# Autodesk Inventor assembly: Julie
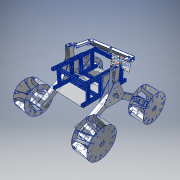
[picture p0: Inventor's stored thumbnail of the model, 180x180]
Saved by Autodesk Inventor 2019 (Build 230136000, 136)
## iProperties
Created: 2018-09-27
Part Number: Julie
Document SubType Name: Assembly
Designer: Adhik
Mass: 21285.8 g
Surface Area: 63277.1 cm^2
Volume: 8790.97 cm^3
Density: 2.42133 g/cm^3
Author: Adhik
## Documents named in this file (19)
- C:\Users\Adhik\Documents\CAD\Julie\Julie.iam
- C:\Users\Adhik\Documents\CAD\Julie\Baseplate.ipt
- C:\Users\Adhik\Documents\CAD\Julie\Lateral Plate.ipt
- C:\Users\Adhik\Documents\CAD\Julie\Right Drive Assembly.iam
- C:\Users\Adhik\Documents\CAD\Julie\Main Joint.ipt
- C:\Users\Adhik\Documents\CAD\Julie\8020 20 inch lower.ipt
- C:\Users\Adhik\Documents\CAD\Julie\8020 6 inch.ipt
- C:\Users\Adhik\Documents\CAD\Julie\Main Axle.ipt
- C:\Users\Adhik\Documents\CAD\Julie\8020 12 inch.ipt
- C:\Users\Adhik\Documents\CAD\Julie\Clamp Collar.ipt
- C:\Users\Adhik\Documents\CAD\Julie\Coupler.ipt
- C:\Users\Adhik\Documents\CAD\Julie\Crossbeam Bearing Mount.ipt
- C:\Users\Adhik\Documents\CAD\Julie\Joint Mount.ipt
- C:\Users\Adhik\Documents\CAD\Julie\Ball Joint.ipt
- C:\Users\Adhik\Documents\CAD\Julie\Crossbeam.ipt
- C:\Users\Adhik\Documents\CAD\Julie\Crossbeam Post.ipt
- C:\Users\Adhik\Documents\CAD\Julie\Front Cover.ipt
- C:\Users\Adhik\Documents\CAD\Julie\Rear Cover.ipt
- C:\Users\Adhik\Documents\CAD\Julie\8020 20 inch upper.ipt
## Components (40 placed, 18 different names)
1. Baseplate:1 — Flush:5, Flush:6, Mate:13, Mate:14, Mate:15, Mate:16, Mate:35, Mate:36, Flush:34, Flush:35
2. Lateral Plate:1 — Flush:5, Mate:5, Mate:7, Mate:8, Mate:14, Mate:18, Mate:23, Mate:24, Mate:86, Mate:87, Mate:88, Mate:89, Flush:28, Flush:30, Flush:31
3. Lateral Plate:2 — Flush:6, Mate:6, Mate:9, Mate:10, Mate:13, Mate:17, Mate:21, Mate:22, Flush:27, Flush:32, Flush:33
4. Right Drive Assembly:2 [sub-assembly] — Mate:11, Mate:34, Mate:50, Mate:58, Mate:60, Mate:61
5. Main Joint:1 — Mate:5, Mate:7, Mate:8, Mate:56
6. Main Joint:2 — Mate:6, Mate:9, Mate:10, Mate:11, Mate:32, Mate:34
7. 8020 20 inch lower:1 — Mate:15, Mate:17, Mate:25, Mate:26, Mate:37, Mate:39, Mate:90, Flush:23, Mate:91, Flush:24, Flush:35, Flush:36
8. 8020 20 inch lower:2 — Mate:16, Mate:18, Mate:27, Mate:28, Mate:92, Mate:93, Flush:25, Flush:26, Flush:34, Flush:39
9. 8020 6 inch:1 — Mate:21, Mate:25, Mate:46, Mate:98, Flush:37
10. 8020 6 inch:2 — Mate:22, Mate:26, Mate:44
11. 8020 6 inch:3 — Mate:24, Mate:27
12. 8020 6 inch:4 — Mate:23, Mate:28, Flush:38, Mate:99
13. Main Axle:1 — Mate:31, Mate:32, Mate:48, Mate:49, Mate:55
14. 8020 12 inch:1 — Mate:35, Mate:37
15. 8020 12 inch:2 — Mate:36, Mate:39, Mate:97
16. 8020 12 inch:3 — Mate:44, Mate:53, Mate:54, Flush:21, Flush:22, Mate:101
17. 8020 12 inch:4 — Mate:46, Flush:40, Mate:100
18. Clamp Collar:1 — Mate:48, Mate:50
19. Clamp Collar:2 — Mate:49, Mate:57
20. Coupler:1 — Mate:72, Mate:79
21. Coupler:2 — Mate:71, Mate:78
22. Crossbeam Bearing Mount:1 — Mate:53, Flush:19, Flush:21, Mate:95, Mate:96
23. Crossbeam Bearing Mount:2 — Mate:54, Flush:20, Flush:22
24. Right Drive Assembly:3 [sub-assembly] — Mate:55, Mate:56, Mate:57, Mate:59, Mate:62, Mate:63
25. Joint Mount:1 — Mate:59, Mate:62, Mate:63, Mate:64, Mate:68, Mate:69
26. Joint Mount:2 — Mate:58, Mate:60, Mate:61, Mate:65, Mate:67, Mate:70
27. Ball Joint:1 — Mate:64, Mate:68, Mate:69, Mate:71
28. Ball Joint:2 — Mate:65, Mate:67, Mate:70, Mate:72
29. Crossbeam:1 — Mate:74, Mate:75, Mate:76, Mate:77, Mate:80, Mate:81, Mate:94, Mate:96
30. Ball Joint:3 — Mate:75, Mate:76, Mate:79, Mate:80
31. Ball Joint:4 — Mate:74, Mate:77, Mate:78, Mate:81
32. Crossbeam Post:1 — Mate:94, Mate:95
33. Front Cover:1 — Mate:86, Mate:87
34. Rear Cover:1 — Mate:88, Mate:89
35. 8020 6 inch:5 — Mate:90, Flush:23, Flush:32
36. 8020 6 inch:6 — Mate:92, Flush:26, Mate:97, Flush:30
37. 8020 6 inch:8 — Mate:93, Flush:25, Flush:31
38. 8020 6 inch:9 — Mate:91, Flush:24, Flush:33
39. 8020 20 inch upper:1 — Flush:36, Mate:98, Flush:37, Flush:40, Mate:100
40. 8020 20 inch upper:2 — Flush:38, Mate:99, Flush:39, Mate:101
## Relationships (99: Mate 76, Flush 23)
- Flush:5: Baseplate:1 ↔ Lateral Plate:1
- Flush:6: Baseplate:1 ↔ Lateral Plate:2
- Mate:5: Lateral Plate:1 ↔ Main Joint:1
- Mate:6: Lateral Plate:2 ↔ Main Joint:2
- Mate:7: Lateral Plate:1 ↔ Main Joint:1
- Mate:8: Lateral Plate:1 ↔ Main Joint:1
- Mate:9: Lateral Plate:2 ↔ Main Joint:2
- Mate:10: Lateral Plate:2 ↔ Main Joint:2
- Mate:11: Right Drive Assembly:2 ↔ Main Joint:2
- Mate:13: Baseplate:1 ↔ Lateral Plate:2
- Mate:14: Baseplate:1 ↔ Lateral Plate:1
- Mate:15: Baseplate:1 ↔ 8020 20 inch lower:1
- Mate:16: Baseplate:1 ↔ 8020 20 inch lower:2
- Mate:17: Lateral Plate:2 ↔ 8020 20 inch lower:1
- Mate:18: Lateral Plate:1 ↔ 8020 20 inch lower:2
- Mate:21: Lateral Plate:2 ↔ 8020 6 inch:1
- Mate:22: Lateral Plate:2 ↔ 8020 6 inch:2
- Mate:23: Lateral Plate:1 ↔ 8020 6 inch:4
- Mate:24: Lateral Plate:1 ↔ 8020 6 inch:3
- Mate:25: 8020 20 inch lower:1 ↔ 8020 6 inch:1
- Mate:26: 8020 20 inch lower:1 ↔ 8020 6 inch:2
- Mate:27: 8020 20 inch lower:2 ↔ 8020 6 inch:3
- Mate:28: 8020 20 inch lower:2 ↔ 8020 6 inch:4
- Mate:31: Main Axle:1
- Mate:32: Main Joint:2 ↔ Main Axle:1
- Mate:34: Right Drive Assembly:2 ↔ Main Joint:2
- Mate:35: Baseplate:1 ↔ 8020 12 inch:1
- Mate:36: Baseplate:1 ↔ 8020 12 inch:2
- Mate:37: 8020 20 inch lower:1 ↔ 8020 12 inch:1
- Mate:39: 8020 20 inch lower:1 ↔ 8020 12 inch:2
- Mate:44: 8020 6 inch:2 ↔ 8020 12 inch:3
- Mate:46: 8020 6 inch:1 ↔ 8020 12 inch:4
- Mate:48: Main Axle:1 ↔ Clamp Collar:1
- Mate:49: Main Axle:1 ↔ Clamp Collar:2
- Mate:50: Right Drive Assembly:2 ↔ Clamp Collar:1
- Mate:53: 8020 12 inch:3 ↔ Crossbeam Bearing Mount:1
- Mate:54: 8020 12 inch:3 ↔ Crossbeam Bearing Mount:2
- Flush:19: Crossbeam Bearing Mount:1
- Flush:20: Crossbeam Bearing Mount:2
- Flush:21: 8020 12 inch:3 ↔ Crossbeam Bearing Mount:1
- Flush:22: 8020 12 inch:3 ↔ Crossbeam Bearing Mount:2
- Mate:55: Main Axle:1 ↔ Right Drive Assembly:3
- Mate:56: Main Joint:1 ↔ Right Drive Assembly:3
- Mate:57: Clamp Collar:2 ↔ Right Drive Assembly:3
- Mate:58: Right Drive Assembly:2 ↔ Joint Mount:2
- Mate:59: Right Drive Assembly:3 ↔ Joint Mount:1
- Mate:60: Right Drive Assembly:2 ↔ Joint Mount:2
- Mate:61: Right Drive Assembly:2 ↔ Joint Mount:2
- Mate:62: Right Drive Assembly:3 ↔ Joint Mount:1
- Mate:63: Right Drive Assembly:3 ↔ Joint Mount:1
- Mate:64: Joint Mount:1 ↔ Ball Joint:1
- Mate:65: Joint Mount:2 ↔ Ball Joint:2
- Mate:67: Joint Mount:2 ↔ Ball Joint:2
- Mate:68: Joint Mount:1 ↔ Ball Joint:1
- Mate:69: Joint Mount:1 ↔ Ball Joint:1
- Mate:70: Joint Mount:2 ↔ Ball Joint:2
- Mate:71: Coupler:2 ↔ Ball Joint:1
- Mate:72: Coupler:1 ↔ Ball Joint:2
- Mate:74: Crossbeam:1 ↔ Ball Joint:4
- Mate:75: Crossbeam:1 ↔ Ball Joint:3
- Mate:76: Crossbeam:1 ↔ Ball Joint:3
- Mate:77: Crossbeam:1 ↔ Ball Joint:4
- Mate:78: Coupler:2 ↔ Ball Joint:4
- Mate:79: Coupler:1 ↔ Ball Joint:3
- Mate:80: Crossbeam:1 ↔ Ball Joint:3
- Mate:81: Crossbeam:1 ↔ Ball Joint:4
- Mate:86: Lateral Plate:1 ↔ Front Cover:1
- Mate:87: Lateral Plate:1 ↔ Front Cover:1
- Mate:88: Lateral Plate:1 ↔ Rear Cover:1
- Mate:89: Lateral Plate:1 ↔ Rear Cover:1
- Mate:90: 8020 20 inch lower:1 ↔ 8020 6 inch:5
- Flush:23: 8020 20 inch lower:1 ↔ 8020 6 inch:5
- Mate:91: 8020 20 inch lower:1 ↔ 8020 6 inch:9
- Flush:24: 8020 20 inch lower:1 ↔ 8020 6 inch:9
- Mate:92: 8020 20 inch lower:2 ↔ 8020 6 inch:6
- Mate:93: 8020 20 inch lower:2 ↔ 8020 6 inch:8
- Flush:25: 8020 20 inch lower:2 ↔ 8020 6 inch:8
- Flush:26: 8020 20 inch lower:2 ↔ 8020 6 inch:6
- Mate:94: Crossbeam:1 ↔ Crossbeam Post:1
- Mate:95: Crossbeam Bearing Mount:1 ↔ Crossbeam Post:1
- Flush:27: Lateral Plate:2
- Flush:28: Lateral Plate:1
- Mate:96 (12.7 mm): Crossbeam Bearing Mount:1 ↔ Crossbeam:1
- Mate:97: 8020 12 inch:2 ↔ 8020 6 inch:6
- Flush:30: Lateral Plate:1 ↔ 8020 6 inch:6
- Flush:31: Lateral Plate:1 ↔ 8020 6 inch:8
- Flush:32: Lateral Plate:2 ↔ 8020 6 inch:5
- Flush:33: Lateral Plate:2 ↔ 8020 6 inch:9
- Flush:34: Baseplate:1 ↔ 8020 20 inch lower:2
- Flush:35: Baseplate:1 ↔ 8020 20 inch lower:1
- Flush:36: 8020 20 inch lower:1 ↔ 8020 20 inch upper:1
- Mate:98: 8020 6 inch:1 ↔ 8020 20 inch upper:1
- Flush:37: 8020 6 inch:1 ↔ 8020 20 inch upper:1
- Flush:38: 8020 6 inch:4 ↔ 8020 20 inch upper:2
- Mate:99: 8020 6 inch:4 ↔ 8020 20 inch upper:2
- Flush:39: 8020 20 inch lower:2 ↔ 8020 20 inch upper:2
- Flush:40: 8020 12 inch:4 ↔ 8020 20 inch upper:1
- Mate:100: 8020 12 inch:4 ↔ 8020 20 inch upper:1
- Mate:101: 8020 12 inch:3 ↔ 8020 20 inch upper:2
